# Autodesk Inventor assembly: Chain Drive
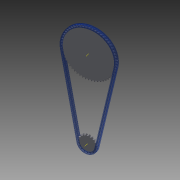
[picture p0: Inventor's stored thumbnail of the model, 180x180]
Saved by Autodesk Inventor 2011 (Build 150239000, 239)
## iProperties
Created: 2011-01-19
Part Number: Chain Drive
Document SubType Name: Assembly
Designer: fcboe
ClientObjectVersion: 1
Author: fcboe
## Documents named in this file (4)
- C:\Users\fcboe\Desktop\Chain Drive2.iam
- C:\Users\fcboe\Desktop\Assembly1\Design Accelerator\Roller Chain2.ipt
- C:\Users\fcboe\Desktop\Assembly1\Design Accelerator\Roller Chain Sprocket11.ipt
- C:\Users\fcboe\Desktop\Assembly1\Design Accelerator\Roller Chain Sprocket22.ipt
## Components (3 placed, 3 different names)
1. Roller Chain:1 — Flush:1, Mate:1, Mate:2, Flush:2, Mate:3, Mate:4
2. Roller Chain Sprocket1:1 — Flush:1, Mate:1, Mate:2, Rotation:1
3. Roller Chain Sprocket2:1 — Flush:2, Mate:3, Rotation:1, Mate:4
## Relationships (7: Mate 4, Flush 2, RelateRotation 1)
- Flush:1: Roller Chain:1 ↔ Roller Chain Sprocket1:1
- Flush:2: Roller Chain:1 ↔ Roller Chain Sprocket2:1
- Rotation:1 [RelateRotation] (3 ul): Roller Chain Sprocket1:1 ↔ Roller Chain Sprocket2:1
- Mate:1: Roller Chain:1 ↔ Roller Chain Sprocket1:1
- Mate:2: Roller Chain:1 ↔ Roller Chain Sprocket1:1
- Mate:3: Roller Chain:1 ↔ Roller Chain Sprocket2:1
- Mate:4: Roller Chain:1 ↔ Roller Chain Sprocket2:1
